# Autodesk Inventor assembly: Assembly Guitarra 2
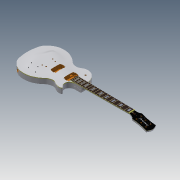
[picture p0: Inventor's stored thumbnail of the model, 180x180]
Saved by Autodesk Inventor 2016 (Build 200138000, 138)
## iProperties
Created: 2018-11-08
Part Number: Assembly Guitarra 2
Document SubType Name: Assembly
Designer: Pedro Mendonça
Author: Pedro Mendonça
## Documents named in this file (5)
- C:\Users\Pedro\Google Drive\Projeto CAD Eng Mecânica\Assembly Guitarra 2.iam
- C:\Users\Pedro\Google Drive\Projeto CAD Eng Mecânica\Corpo.ipt
- C:\Users\Pedro\Google Drive\Projeto CAD Eng Mecânica\Braço.ipt
- C:\Users\Pedro\Google Drive\Projeto CAD Eng Mecânica\Tampo.ipt
- C:\Users\Pedro\Google Drive\Projeto CAD Eng Mecânica\Potenciometro.ipt
## Components (7 placed, 4 different names)
1. Corpo:1 — Cylindrical:2, Cylindrical:3
2. Braço:1 — Cylindrical:2
3. Tampo:1 — Cylindrical:3, Cylindrical:7, Cylindrical:4, Cylindrical:8, Cylindrical:9
4. Potenciometro:1 — Cylindrical:7
5. Potenciometro:2 — Cylindrical:4
6. Potenciometro:3 — Cylindrical:9
7. Potenciometro:4 — Cylindrical:8
## Relationships (6: CylindricalJoint 6)
- Cylindrical:2: Corpo:1 ↔ Braço:1
- Cylindrical:3: Corpo:1 ↔ Tampo:1
- Cylindrical:7: Tampo:1 ↔ Potenciometro:1
- Cylindrical:4: Tampo:1 ↔ Potenciometro:2
- Cylindrical:8: Tampo:1 ↔ Potenciometro:4
- Cylindrical:9: Tampo:1 ↔ Potenciometro:3
